# Autodesk Inventor assembly: Surub M4 saiba piulita
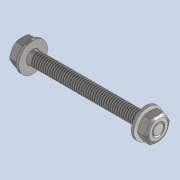
[picture p0: Inventor's stored thumbnail of the model, 180x180]
Saved by Autodesk Inventor 2020 (Build 240168000, 168)
## iProperties
Created: 2020-12-19
Part Number: Surub M4 saiba piulita
Document SubType Name: Assembly
Designer: Iulian Bors
Author: Iulian Bors
## Documents named in this file (4)
- Z:\I.A.B\Proiecte\0005 I.A.B 3d 2.0 Imprimanta aracet\10 Mecanic\Surub M4 saiba piulita.iam
- Z:\I.A.B\Proiecte\0005 I.A.B 3d 2.0 Imprimanta aracet\10 Mecanic\0005-10-1013 ISO 7089 - 4 - 140 HV.ipt
- Z:\I.A.B\Proiecte\0005 I.A.B 3d 2.0 Imprimanta aracet\10 Mecanic\0005-10-1014 ISO 4032 - M4 - ISO.ipt
- Z:\I.A.B\Proiecte\0005 I.A.B 3d 2.0 Imprimanta aracet\10 Mecanic\0005-10-1024 ISO 4017 - M4 x 40 - ISO copy.ipt
## Components (4 placed, 3 different names)
1. 0005-10-1024 ISO 4017 - M4 x 40 - ISO copy.ipt:1
2. 0005-10-1013 ISO 7089 - 4 - 140 HV.ipt:2
3. 0005-10-1014 ISO 4032 - M4 - ISO.ipt:3 — Insert:1
4. 0005-10-1013 ISO 7089 - 4 - 140 HV.ipt:4 — Insert:1
## Relationships (4: Mate 2, Insert 2)
- [Mate]: 0005-10-1024 ISO 4017 - M4 x 40 - ISO copy.ipt:1 ↔ 0005-10-1013 ISO 7089 - 4 - 140 HV.ipt:2
- [Mate]: 0005-10-1024 ISO 4017 - M4 x 40 - ISO copy.ipt:1 ↔ 0005-10-1013 ISO 7089 - 4 - 140 HV.ipt:2
- Insert:1: 0005-10-1014 ISO 4032 - M4 - ISO.ipt:3 ↔ 0005-10-1013 ISO 7089 - 4 - 140 HV.ipt:4
- [Insert]: 0005-10-1024 ISO 4017 - M4 x 40 - ISO copy.ipt:1 ↔ 0005-10-1014 ISO 4032 - M4 - ISO.ipt:3
